# Autodesk Inventor assembly: Spincoater Assem
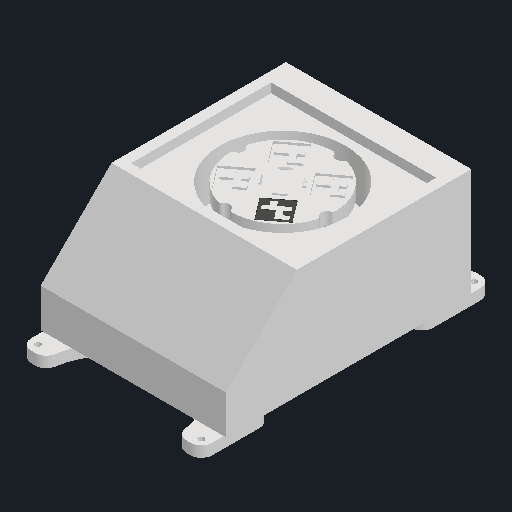
[picture p0: Inventor's stored thumbnail of the model, 512x512]
Saved by Autodesk Inventor 2026 (Build 300175000, 175)
## iProperties
Created: 2025-02-26
Part Number: Spincoater Assem
Document SubType Name: Assembly
Designer: jerem
Author: jerem
## Documents named in this file (4)
- C:\Users\jerem\Documents\GitHub\Perovskite-Automated-Synthesis-System\CAD\Spin-Chuck\Spincoater Assem.iam
- C:\Users\jerem\Documents\GitHub\Perovskite-Automated-Synthesis-System\CAD\Non 3D Printed Parts\Spin Coater.ipt
- C:\Users\jerem\Documents\GitHub\Perovskite-Automated-Synthesis-System\CAD\Object Mounts\Spincoater Base Mount.ipt
- C:\Users\jerem\Documents\GitHub\Perovskite-Automated-Synthesis-System\CAD\Spin-Chuck\Spin Chuck.ipt
## Components (3 placed, 3 different names)
1. Spin Coater:1 — Mate:4, Flush:1
2. Spincoater Base Mount:1
3. Spin Chuck:1 — Mate:4, Flush:1
## Relationships (5: Mate 4, Flush 1)
- [Mate]: Spin Coater:1 ↔ Spincoater Base Mount:1
- [Mate]: Spin Coater:1 ↔ Spincoater Base Mount:1
- [Mate]: Spin Coater:1 ↔ Spincoater Base Mount:1
- Mate:4: Spin Coater:1 ↔ Spin Chuck:1
- Flush:1: Spin Coater:1 ↔ Spin Chuck:1
